# Autodesk Inventor assembly: plate_assembly_stacked
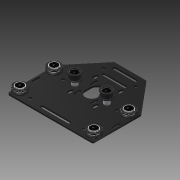
[picture p0: Inventor's stored thumbnail of the model, 180x180]
Saved by Autodesk Inventor 2014 (Build 180170000, 170)
## iProperties
Created: 2013-05-29
Part Number: plate_assembly_stacked
Document SubType Name: Assembly
Designer: Edward
Mass: 864.739 g
Surface Area: 894.967 cm^2
Volume: 163.574 cm^3
Density: 5.28654 g/cm^3
Author: Edward
## Documents named in this file (10)
- C:\Users\Edward\Documents\Vault\Designs\Shapeoko_v2\v2_final\plate_assembly_stacked.iam
- C:\Users\Edward\Documents\Vault\Designs\Shapeoko_v2\v2_final\26029-01.ipt
- C:\Users\Edward\Documents\Vault\Designs\Shapeoko_v2\v2_final\B18033.ipt
- C:\Users\Edward\Documents\Vault\Designs\Shapeoko_v2\v2_final\25203-02.iam
- C:\Users\Edward\Documents\Vault\Designs\Shapeoko_v2\v2_final\91239A233.ipt
- C:\Users\Edward\Documents\Vault\Designs\Shapeoko_v2\v2_final\25287-02.ipt
- C:\Users\Edward\Documents\Vault\Designs\Shapeoko_v2\v2_final\25284-02.ipt
- C:\Users\Edward\Documents\Vault\Designs\Shapeoko_v2\v2_final\25197-02.iam
- C:\Users\Edward\Documents\Vault\Designs\Shapeoko_v2\v2_final\25286-05.ipt
- C:\Users\Edward\Documents\Vault\Designs\Shapeoko_v2\v2_final\25312-14.ipt
## Components (33 placed, 9 different names)
1. 26029-01:1 — Insert:3, Insert:5, Insert:9, Mate:2, Insert:10, Mate:4, Insert:15, Insert:16, Insert:21, Insert:24, Insert:26, Insert:43
2. B18033:1 — Insert:10, Mate:3
3. B18033:2 — Mate:1, Insert:9
4. 25203-02:4 [sub-assembly] — Insert:2, Insert:4
5. 25287-02:1 — Insert:2, Insert:3
6. 91239A233:2 — Insert:4
7. 25287-02:2 — Insert:11, Mate:4
8. 25284-02:2 — Insert:6
9. 25287-02:4 — Insert:16, Insert:17
10. 25287-02:5 — Insert:14, Insert:15
11. 25287-02:6 — Insert:7, Mate:2
12. 25287-02:7 — Insert:5, Insert:6
13. 91239A233:3 — Insert:8, Mate:1
14. 25203-02:5 [sub-assembly] — Insert:7, Insert:8
15. 91239A233:4 — Insert:12, Mate:3
16. 25203-02:6 [sub-assembly] — Insert:11, Insert:12
17. 91239A233:5 — Insert:13
18. 25203-02:7 [sub-assembly] — Insert:13, Insert:14
19. 25284-02:3 — Insert:17
20. 25197-02:1 [sub-assembly]
21. 25197-02:2 [sub-assembly] — Insert:21
22. 25286-05:2
23. 25287-02:8 — Insert:23, Insert:24
24. 25284-02:4 — Insert:23
25. 25286-05:1
26. 25284-02:5 — Insert:27
27. 25287-02:9 — Insert:26, Insert:27
28. 25312-14:1 — Insert:39
29. 25312-14:2 — Insert:41
30. 25287-02:10 — Insert:39, Insert:40
31. 25287-02:11 — Insert:40
32. 25287-02:12 — Insert:41, Insert:42
33. 25287-02:13 — Insert:42, Insert:43
## Relationships (34: Insert 30, Mate 4)
- Insert:2: 25203-02:4 ↔ 25287-02:1
- Insert:3: 26029-01:1 ↔ 25287-02:1
- Insert:4: 25203-02:4 ↔ 91239A233:2
- Insert:5: 26029-01:1 ↔ 25287-02:7
- Insert:6: 25284-02:2 ↔ 25287-02:7
- Insert:7: 25287-02:6 ↔ 25203-02:5
- Insert:8: 91239A233:3 ↔ 25203-02:5
- Mate:1: B18033:2 ↔ 91239A233:3
- Insert:9: 26029-01:1 ↔ B18033:2
- Mate:2: 26029-01:1 ↔ 25287-02:6
- Insert:10: 26029-01:1 ↔ B18033:1
- Insert:11: 25287-02:2 ↔ 25203-02:6
- Insert:12: 91239A233:4 ↔ 25203-02:6
- Mate:3: B18033:1 ↔ 91239A233:4
- Mate:4: 26029-01:1 ↔ 25287-02:2
- Insert:13: 91239A233:5 ↔ 25203-02:7
- Insert:14: 25287-02:5 ↔ 25203-02:7
- Insert:15: 26029-01:1 ↔ 25287-02:5
- Insert:16: 26029-01:1 ↔ 25287-02:4
- Insert:17: 25287-02:4 ↔ 25284-02:3
- Insert:21 (9.525 mm): 26029-01:1 ↔ 25197-02:2
- [Insert]: 25197-02:1 ↔ 25286-05:2
- Insert:23: 25287-02:8 ↔ 25284-02:4
- Insert:24: 26029-01:1 ↔ 25287-02:8
- [Insert]: 25197-02:2 ↔ 25286-05:1
- Insert:26: 26029-01:1 ↔ 25287-02:9
- Insert:27: 25284-02:5 ↔ 25287-02:9
- [Insert]: 25197-02:2 ↔ 25312-14:1
- [Insert]: 25197-02:1 ↔ 25312-14:2
- Insert:39: 25312-14:1 ↔ 25287-02:10
- Insert:40: 25287-02:10 ↔ 25287-02:11
- Insert:41: 25312-14:2 ↔ 25287-02:12
- Insert:42: 25287-02:12 ↔ 25287-02:13
- Insert:43: 26029-01:1 ↔ 25287-02:13
